# Autodesk Inventor assembly: B
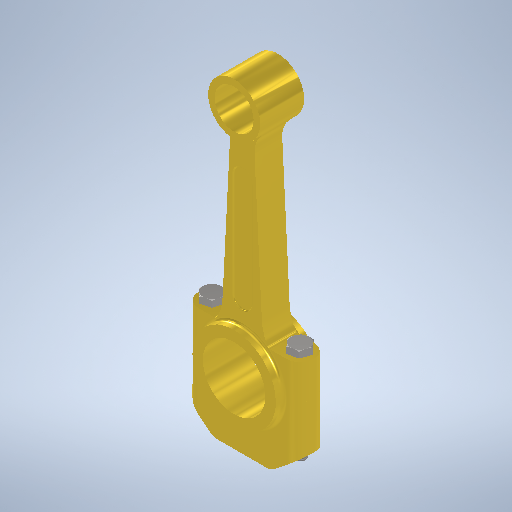
[picture p0: Inventor's stored thumbnail of the model, 512x512]
Saved by Autodesk Inventor 2025.2 (Build 292293000, 293)
## iProperties
Created: 2025-03-20
Part Number: B
Document SubType Name: Assembly
Designer: User
Author: User
## Documents named in this file (5)
- C:\Users\User\Documents\Inventor\Engine\B.iam
- C:\Users\User\Documents\Inventor\Engine\Part 3 Connecting rod.ipt
- C:\Users\User\Documents\Inventor\Engine\Part 4 Connecting rods cap.ipt
- C:\Users\User\Documents\Inventor\Content Center Files\R2025\en-US\DIN EN ISO 4032\DIN EN ISO 4032 - M10.ipt
- C:\Users\User\Documents\Inventor\Content Center Files\R2025\en-US\BS EN ISO 4017\BS EN ISO 4017 - M10 x 80BS EN.ipt
## Components (6 placed, 4 different names)
1. Part 3 Connecting rod:1 — Mate:1, Mate:2, Mate:3, Mate:4, Mate:5, Mate:6, Mate:7
2. Part 4 Connecting rods cap:1 — Mate:1, Mate:2, Mate:3, Mate:10, Mate:11
3. DIN EN ISO 4032 M10:1 — Mate:8, Mate:10
4. DIN EN ISO 4032 M10:2 — Mate:9, Mate:11
5. BS EN ISO 4017 - Metric M10 x 80:1 — Mate:6, Mate:7, Mate:8
6. BS EN ISO 4017 - Metric M10 x 80:2 — Mate:4, Mate:5, Mate:9
## Relationships (11: Mate 11)
- Mate:1: Part 3 Connecting rod:1 ↔ Part 4 Connecting rods cap:1
- Mate:2: Part 3 Connecting rod:1 ↔ Part 4 Connecting rods cap:1
- Mate:3: Part 3 Connecting rod:1 ↔ Part 4 Connecting rods cap:1
- Mate:4: Part 3 Connecting rod:1 ↔ BS EN ISO 4017 - Metric M10 x 80:2
- Mate:5: Part 3 Connecting rod:1 ↔ BS EN ISO 4017 - Metric M10 x 80:2
- Mate:6: Part 3 Connecting rod:1 ↔ BS EN ISO 4017 - Metric M10 x 80:1
- Mate:7: Part 3 Connecting rod:1 ↔ BS EN ISO 4017 - Metric M10 x 80:1
- Mate:8: DIN EN ISO 4032 M10:1 ↔ BS EN ISO 4017 - Metric M10 x 80:1
- Mate:9: DIN EN ISO 4032 M10:2 ↔ BS EN ISO 4017 - Metric M10 x 80:2
- Mate:10: Part 4 Connecting rods cap:1 ↔ DIN EN ISO 4032 M10:1
- Mate:11: Part 4 Connecting rods cap:1 ↔ DIN EN ISO 4032 M10:2
